# Autodesk Inventor assembly: X_CarriageFWD_V2_1
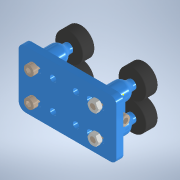
[picture p0: Inventor's stored thumbnail of the model, 180x180]
Saved by Autodesk Inventor 2022 (Build 260153000, 153)
## iProperties
Created: 2021-06-13
Part Number: X_CarriageFWD_V2_1
Document SubType Name: Assembly
Designer: Jorian Brusind
Author: Jorian Brusind
## Documents named in this file (8)
- C:\Users\Jorian Brusind\Documents\GitHub\HyperRail\Inventor Files\X_CarriageFWD_V2_1.iam
- C:\Users\Jorian Brusind\Documents\GitHub\HyperRail\Inventor Files\X_Carriage_Plate.ipt
- C:\Users\Jorian Brusind\Documents\GitHub\HyperRail\Inventor Files\11mm_BearingWheel.ipt
- C:\Users\Jorian Brusind\Documents\GitHub\HyperRail\Inventor Files\4mm_Roller_Spacer_simple.ipt
- C:\Users\Jorian Brusind\Documents\GitHub\HyperRail\Inventor Files\Metric Spacer_Standoffs\hex spacer standoff nut M5 L30.ipt
- C:\Users\Jorian Brusind\Documents\GitHub\HyperRail\Inventor Files\Metric bolt\Bolt M5 30mm.ipt
- C:\Users\Jorian Brusind\Documents\GitHub\HyperRail\Inventor Files\Metric bolt\Bolt M5 45mm.ipt
- C:\Users\Jorian Brusind\Documents\GitHub\HyperRail\Inventor Files\Metric nuts\Nut M5.ipt
## Components (16 placed, 7 different names)
1. X_Carriage_Plate:1 — Mate:14, Mate:33, Mate:42, Angle:1, Angle:2, Mate:45, Mate:62, Mate:63, Mate:66
2. 11mm_BearingWheel:1 — Flush:2, Mate:43, Mate:49, Mate:58, Mate:60
3. 11mm_BearingWheel:4 — Flush:2, Mate:44, Mate:59, Mate:61
4. 4mm_Roller_Spacer_simple:2 — Mate:14, Mate:42, Angle:1, Mate:46, Mate:47, Mate:48, Mate:50, Mate:55, Mate:56, Mate:57
5. 4mm_Roller_Spacer_simple:3 — Mate:33, Mate:43, Mate:44, Angle:2, Mate:45, Mate:49, Mate:52, Mate:53, Mate:54
6. 11mm_BearingWheel:5 — Mate:46, Flush:3, Mate:48
7. 11mm_BearingWheel:6 — Mate:47, Flush:3
8. hex spacer standoff nut M5 L30:1 — Mate:51, Mate:53
9. Bolt M5 30mm:1 — Mate:52, Mate:54
10. Bolt M5 30mm:2 — Mate:50, Mate:51, Mate:55
11. Bolt M5 45mm:1 — Mate:57, Mate:62
12. Bolt M5 45mm:2 — Mate:56, Mate:63
13. Bolt M5 45mm:3 — Mate:59, Mate:61, Mate:64
14. Bolt M5 45mm:4 — Mate:58, Mate:60, Mate:65
15. Nut M5:1 — Mate:64, Flush:4
16. Nut M5:2 — Mate:65, Flush:4, Mate:66
## Relationships (32: Mate 27, Flush 3, Angle 2)
- Flush:2: 11mm_BearingWheel:1 ↔ 11mm_BearingWheel:4
- Mate:14: X_Carriage_Plate:1 ↔ 4mm_Roller_Spacer_simple:2
- Mate:33: X_Carriage_Plate:1 ↔ 4mm_Roller_Spacer_simple:3
- Mate:42 (-12.5 mm): X_Carriage_Plate:1 ↔ 4mm_Roller_Spacer_simple:2
- Angle:1 (0 deg): X_Carriage_Plate:1 ↔ 4mm_Roller_Spacer_simple:2
- Mate:43: 11mm_BearingWheel:1 ↔ 4mm_Roller_Spacer_simple:3
- Mate:44: 11mm_BearingWheel:4 ↔ 4mm_Roller_Spacer_simple:3
- Angle:2 (0 deg): X_Carriage_Plate:1 ↔ 4mm_Roller_Spacer_simple:3
- Mate:45 (-12.5 mm): X_Carriage_Plate:1 ↔ 4mm_Roller_Spacer_simple:3
- Mate:46: 4mm_Roller_Spacer_simple:2 ↔ 11mm_BearingWheel:5
- Mate:47: 4mm_Roller_Spacer_simple:2 ↔ 11mm_BearingWheel:6
- Flush:3: 11mm_BearingWheel:5 ↔ 11mm_BearingWheel:6
- Mate:48: 4mm_Roller_Spacer_simple:2 ↔ 11mm_BearingWheel:5
- Mate:49: 11mm_BearingWheel:1 ↔ 4mm_Roller_Spacer_simple:3
- Mate:50: 4mm_Roller_Spacer_simple:2 ↔ Bolt M5 30mm:2
- Mate:51: hex spacer standoff nut M5 L30:1 ↔ Bolt M5 30mm:2
- Mate:52: 4mm_Roller_Spacer_simple:3 ↔ Bolt M5 30mm:1
- Mate:53 (10 mm): 4mm_Roller_Spacer_simple:3 ↔ hex spacer standoff nut M5 L30:1
- Mate:54: 4mm_Roller_Spacer_simple:3 ↔ Bolt M5 30mm:1
- Mate:55: 4mm_Roller_Spacer_simple:2 ↔ Bolt M5 30mm:2
- Mate:56: 4mm_Roller_Spacer_simple:2 ↔ Bolt M5 45mm:2
- Mate:57: 4mm_Roller_Spacer_simple:2 ↔ Bolt M5 45mm:1
- Mate:58: 11mm_BearingWheel:1 ↔ Bolt M5 45mm:4
- Mate:59: 11mm_BearingWheel:4 ↔ Bolt M5 45mm:3
- Mate:60: 11mm_BearingWheel:1 ↔ Bolt M5 45mm:4
- Mate:61: 11mm_BearingWheel:4 ↔ Bolt M5 45mm:3
- Mate:62: X_Carriage_Plate:1 ↔ Bolt M5 45mm:1
- Mate:63: X_Carriage_Plate:1 ↔ Bolt M5 45mm:2
- Mate:64: Bolt M5 45mm:3 ↔ Nut M5:1
- Mate:65: Bolt M5 45mm:4 ↔ Nut M5:2
- Flush:4: Nut M5:1 ↔ Nut M5:2
- Mate:66: X_Carriage_Plate:1 ↔ Nut M5:2
